# Autodesk Inventor assembly: phone-stand-assembly
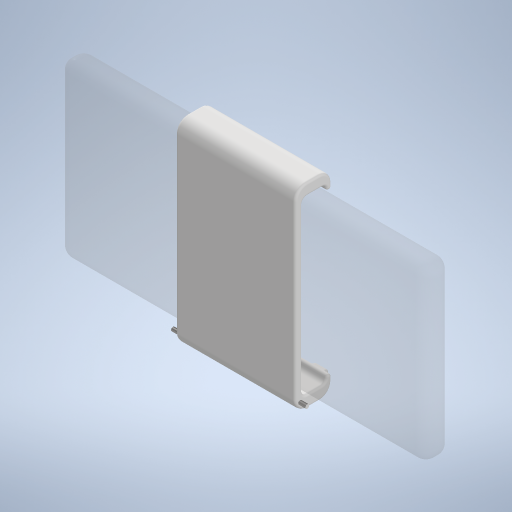
[picture p0: Inventor's stored thumbnail of the model, 512x512]
Saved by Autodesk Inventor 2023 (Build 270158030, 158C)
## iProperties
Created: 2023-04-28
Part Number: phone-stand-assembly
Document SubType Name: Assembly
Designer: Imogen Heard
Author: Imogen Heard
## Documents named in this file (4)
- C:\Users\dheard\Documents\0004-inventor\3D_CAD_Master\phone-holder\phone-stand-assembly.iam
- C:\Users\dheard\Documents\0004-inventor\3D_CAD_Master\phone-holder\samsung-s20.ipt
- C:\Users\dheard\Documents\0004-inventor\3D_CAD_Master\phone-holder\s20-phone-clip.ipt
- C:\Users\dheard\Documents\0004-inventor\3D_CAD_Master\phone-holder\pin.ipt
## Components (3 placed, 3 different names)
1. samsung-s20:1 — Flush:1, Flush:2
2. s20-phone-clip:1 — Flush:1, Flush:2, Flush:3, Flush:4
3. pin:1 — Flush:3, Flush:4
## Relationships (4: Flush 4)
- Flush:1: samsung-s20:1 ↔ s20-phone-clip:1
- Flush:2: samsung-s20:1 ↔ s20-phone-clip:1
- Flush:3: s20-phone-clip:1 ↔ pin:1
- Flush:4: s20-phone-clip:1 ↔ pin:1
